# Autodesk Inventor assembly: Plataforma_robots
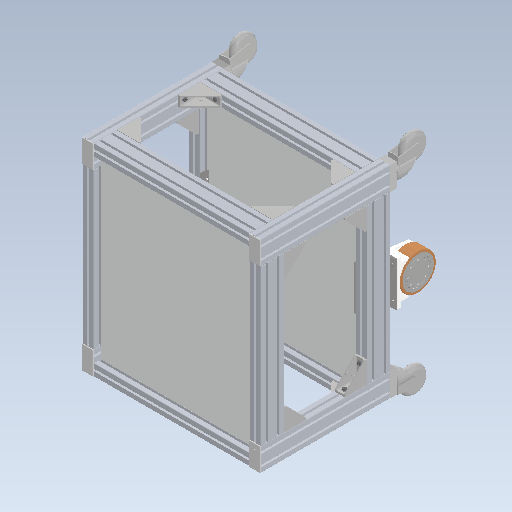
[picture p0: Inventor's stored thumbnail of the model, 512x512]
Saved by Autodesk Inventor 2021 (Build 250183000, 183)
## iProperties
Created: 2020-10-29
Part Number: Plataforma_robots
Document SubType Name: Assembly
Designer: German Di Fonzo
Author: German Di Fonzo
Title: Plataforma para Robots
## Documents named in this file (11)
- C:\Users\germi\OneDrive - Universidad Politécnica de Madrid\Escritorio\German Universidad\Master\Primer semestre\Diseño y Control de Robots\PECs\plataforma_robot\Plataforma_robots.iam
- C:\Users\germi\OneDrive - Universidad Politécnica de Madrid\Escritorio\German Universidad\Master\Primer semestre\Diseño y Control de Robots\PECs\plataforma_robot\Steps\perfil_45x90x600.ipt
- C:\Users\germi\OneDrive - Universidad Politécnica de Madrid\Escritorio\German Universidad\Master\Primer semestre\Diseño y Control de Robots\PECs\plataforma_robot\Steps\perfil_45x90x500.ipt
- C:\Users\germi\OneDrive - Universidad Politécnica de Madrid\Escritorio\German Universidad\Master\Primer semestre\Diseño y Control de Robots\PECs\plataforma_robot\piso1.ipt
- C:\Users\germi\OneDrive - Universidad Politécnica de Madrid\Escritorio\German Universidad\Master\Primer semestre\Diseño y Control de Robots\PECs\plataforma_robot\piso2.ipt
- C:\Users\germi\OneDrive - Universidad Politécnica de Madrid\Escritorio\German Universidad\Master\Primer semestre\Diseño y Control de Robots\PECs\plataforma_robot\Pletina (1).ipt
- C:\Users\germi\OneDrive - Universidad Politécnica de Madrid\Escritorio\German Universidad\Master\Primer semestre\Diseño y Control de Robots\PECs\plataforma_robot\Steps\tapa_superior.ipt
- C:\Users\germi\OneDrive - Universidad Politécnica de Madrid\Escritorio\German Universidad\Master\Primer semestre\Diseño y Control de Robots\PECs\plataforma_robot\Steps\L_45x90.ipt
- C:\Users\germi\OneDrive - Universidad Politécnica de Madrid\Escritorio\German Universidad\Master\Primer semestre\Diseño y Control de Robots\PECs\plataforma_robot\Steps\rueda_motriz.ipt
- C:\Users\germi\OneDrive - Universidad Politécnica de Madrid\Escritorio\German Universidad\Master\Primer semestre\Diseño y Control de Robots\PECs\plataforma_robot\Steps\castor.ipt
- C:\Users\germi\OneDrive - Universidad Politécnica de Madrid\Escritorio\German Universidad\Master\Primer semestre\Diseño y Control de Robots\PECs\plataforma_robot\sujecion_castor.ipt
## Components (46 placed, 10 different names)
1. perfil_45x90x600:1 — Coincidencia:1, Nivelación:1, Nivelación:2, Coincidencia:8, Nivelación:16, Nivelación:17, Coincidencia:19, Nivelación:38, Coincidencia:25, Nivelación:42, Coincidencia:45, Coincidencia:47
2. perfil_45x90x600:2 — Coincidencia:5, Nivelación:9, Nivelación:10, Coincidencia:7, Nivelación:14, Nivelación:15, Coincidencia:20, Nivelación:40, Coincidencia:22, Nivelación:41, Coincidencia:37, Coincidencia:49
3. perfil_45x90x600:3 — Coincidencia:9, Coincidencia:10, Nivelación:18, Nivelación:19, Nivelación:20, Nivelación:21, Nivelación:39, Coincidencia:41, Coincidencia:43
4. perfil_45x90x600:4 — Coincidencia:2, Nivelación:3, Nivelación:4, Nivelación:12, Coincidencia:6, Nivelación:13, Coincidencia:21, Coincidencia:39, Coincidencia:51
5. perfil_45x90x500:1 — Coincidencia:5, Nivelación:9, Nivelación:10, Coincidencia:9, Nivelación:18, Nivelación:21, Coincidencia:12, Nivelación:22, Nivelación:25, Coincidencia:17, Nivelación:34, Nivelación:36, Coincidencia:33, Nivelación:46, Nivelación:47, Coincidencia:40, Nivelación:54, Coincidencia:48, Nivelación:58, Coincidencia:55, Nivelación:61, Coincidencia:56, Nivelación:62, Coincidencia:74, Nivelación:78, Nivelación:79
6. perfil_45x90x500:2 — Coincidencia:8, Nivelación:16, Nivelación:17, Coincidencia:10, Nivelación:19, Nivelación:20, Coincidencia:14, Nivelación:26, Nivelación:29, Coincidencia:18, Nivelación:35, Nivelación:37, Coincidencia:34, Nivelación:48, Nivelación:49, Coincidencia:42, Nivelación:55, Coincidencia:46, Nivelación:57, Coincidencia:59, Nivelación:63, Coincidencia:63, Nivelación:65, Coincidencia:72, Nivelación:74, Nivelación:75
7. perfil_45x90x500:3 — Coincidencia:1, Nivelación:1, Nivelación:2, Coincidencia:2, Nivelación:3, Nivelación:4, Coincidencia:13, Nivelación:27, Nivelación:28, Coincidencia:16, Nivelación:30, Nivelación:33, Coincidencia:35, Nivelación:50, Nivelación:51, Coincidencia:44, Nivelación:56, Coincidencia:50, Nivelación:59, Coincidencia:60, Nivelación:64, Coincidencia:64, Nivelación:66, Coincidencia:70, Nivelación:72, Nivelación:73
8. perfil_45x90x500:4 — Nivelación:12, Coincidencia:6, Nivelación:13, Coincidencia:7, Nivelación:14, Nivelación:15, Coincidencia:11, Nivelación:23, Nivelación:24, Coincidencia:15, Nivelación:31, Nivelación:32, Coincidencia:32, Nivelación:44, Nivelación:45, Coincidencia:36, Nivelación:52, Coincidencia:38, Nivelación:53, Coincidencia:52, Coincidencia:66, Nivelación:67, Coincidencia:73, Nivelación:76, Nivelación:77
9. perfil_45x90x600:5 — Coincidencia:15, Coincidencia:16, Nivelación:30, Nivelación:31, Nivelación:32, Nivelación:33, Coincidencia:31, Coincidencia:65, Coincidencia:67
10. perfil_45x90x600:6 — Coincidencia:13, Coincidencia:14, Nivelación:26, Nivelación:27, Nivelación:28, Nivelación:29, Coincidencia:28, Coincidencia:61, Coincidencia:62
11. perfil_45x90x600:7 — Coincidencia:11, Coincidencia:12, Nivelación:22, Nivelación:23, Nivelación:24, Nivelación:25, Coincidencia:29, Nivelación:43, Coincidencia:53, Nivelación:60, Coincidencia:54
12. perfil_45x90x600:8 — Coincidencia:17, Coincidencia:18, Nivelación:34, Nivelación:35, Nivelación:36, Nivelación:37, Coincidencia:30, Coincidencia:57, Coincidencia:58
13. piso1:2 — Coincidencia:19, Coincidencia:20, Nivelación:38, Nivelación:39, Nivelación:40, Coincidencia:21, Coincidencia:23, Coincidencia:24, Coincidencia:26, Coincidencia:27
14. piso2:3 — Coincidencia:28, Coincidencia:29, Coincidencia:30, Coincidencia:31, Nivelación:43
15. Pletina (1):1 — Coincidencia:22, Coincidencia:23, Coincidencia:24, Nivelación:41, Coincidencia:69, Nivelación:70, Nivelación:71
16. Pletina (1):2 — Coincidencia:25, Coincidencia:26, Coincidencia:27, Nivelación:42, Coincidencia:68, Nivelación:68, Nivelación:69
17. tapa_superior:1 — Coincidencia:32, Nivelación:44, Nivelación:45
18. tapa_superior:2 — Coincidencia:33, Nivelación:46, Nivelación:47
19. tapa_superior:3 — Coincidencia:34, Nivelación:48, Nivelación:49
20. tapa_superior:4 — Coincidencia:35, Nivelación:50, Nivelación:51
21. L_45x90:1 — Coincidencia:46, Nivelación:57, Coincidencia:47
22. L_45x90:2 — Coincidencia:44, Coincidencia:45, Nivelación:56
23. L_45x90:3 — Coincidencia:50, Coincidencia:51, Nivelación:59
24. L_45x90:4 — Coincidencia:38, Coincidencia:39, Nivelación:53
25. L_45x90:5 — Coincidencia:36, Coincidencia:37, Nivelación:52
26. L_45x90:6 — Coincidencia:48, Coincidencia:49, Nivelación:58
27. L_45x90:7 — Coincidencia:40, Coincidencia:41, Nivelación:54
28. L_45x90:8 — Coincidencia:42, Coincidencia:43, Nivelación:55
29. L_45x90:9 — Coincidencia:62, Coincidencia:63, Nivelación:65
30. L_45x90:10 — Coincidencia:54, Coincidencia:55, Nivelación:61
31. L_45x90:11 — Coincidencia:60, Coincidencia:61, Nivelación:64
32. L_45x90:12 — Coincidencia:52, Coincidencia:53, Nivelación:60
33. L_45x90:13 — Coincidencia:56, Coincidencia:57, Nivelación:62
34. L_45x90:14 — Coincidencia:66, Coincidencia:67, Nivelación:67
35. L_45x90:15 — Coincidencia:58, Coincidencia:59, Nivelación:63
36. L_45x90:16 — Coincidencia:64, Coincidencia:65, Nivelación:66
37. rueda_motriz:1 — Coincidencia:69, Nivelación:70, Nivelación:71
38. rueda_motriz:2 — Coincidencia:68, Nivelación:68, Nivelación:69
39. sujecion_castor:1 — Coincidencia:70, Nivelación:72, Nivelación:73, De rotación:1
40. sujecion_castor:2 — Coincidencia:72, Nivelación:74, Nivelación:75, De rotación:2
41. sujecion_castor:3 — Coincidencia:74, Nivelación:78, Nivelación:79, De rotación:4
42. sujecion_castor:4 — Coincidencia:73, Nivelación:76, Nivelación:77, De rotación:3
43. castor:1 — De rotación:1
44. castor:2 — De rotación:3
45. castor:3 — De rotación:4
46. castor:4 — De rotación:2
## Relationships (149: Flush 74, Mate 71, RevoluteJoint 4)
- Coincidencia:1 [Mate]: perfil_45x90x600:1 ↔ perfil_45x90x500:3
- Nivelación:1 [Flush]: perfil_45x90x600:1 ↔ perfil_45x90x500:3
- Nivelación:2 [Flush]: perfil_45x90x600:1 ↔ perfil_45x90x500:3
- Coincidencia:2 [Mate]: perfil_45x90x600:4 ↔ perfil_45x90x500:3
- Nivelación:3 [Flush]: perfil_45x90x600:4 ↔ perfil_45x90x500:3
- Nivelación:4 [Flush]: perfil_45x90x600:4 ↔ perfil_45x90x500:3
- Coincidencia:5 [Mate]: perfil_45x90x600:2 ↔ perfil_45x90x500:1
- Nivelación:9 [Flush]: perfil_45x90x600:2 ↔ perfil_45x90x500:1
- Nivelación:10 [Flush]: perfil_45x90x600:2 ↔ perfil_45x90x500:1
- Nivelación:12 [Flush]: perfil_45x90x600:4 ↔ perfil_45x90x500:4
- Coincidencia:6 [Mate]: perfil_45x90x600:4 ↔ perfil_45x90x500:4
- Nivelación:13 [Flush]: perfil_45x90x600:4 ↔ perfil_45x90x500:4
- Coincidencia:7 [Mate]: perfil_45x90x600:2 ↔ perfil_45x90x500:4
- Nivelación:14 [Flush]: perfil_45x90x600:2 ↔ perfil_45x90x500:4
- Nivelación:15 [Flush]: perfil_45x90x600:2 ↔ perfil_45x90x500:4
- Coincidencia:8 [Mate]: perfil_45x90x600:1 ↔ perfil_45x90x500:2
- Nivelación:16 [Flush]: perfil_45x90x600:1 ↔ perfil_45x90x500:2
- Nivelación:17 [Flush]: perfil_45x90x600:1 ↔ perfil_45x90x500:2
- Coincidencia:9 [Mate]: perfil_45x90x600:3 ↔ perfil_45x90x500:1
- Coincidencia:10 [Mate]: perfil_45x90x600:3 ↔ perfil_45x90x500:2
- Nivelación:18 [Flush]: perfil_45x90x600:3 ↔ perfil_45x90x500:1
- Nivelación:19 [Flush]: perfil_45x90x600:3 ↔ perfil_45x90x500:2
- Nivelación:20 [Flush]: perfil_45x90x600:3 ↔ perfil_45x90x500:2
- Nivelación:21 [Flush]: perfil_45x90x600:3 ↔ perfil_45x90x500:1
- Coincidencia:11 [Mate]: perfil_45x90x500:4 ↔ perfil_45x90x600:7
- Coincidencia:12 [Mate]: perfil_45x90x500:1 ↔ perfil_45x90x600:7
- Nivelación:22 [Flush]: perfil_45x90x500:1 ↔ perfil_45x90x600:7
- Nivelación:23 [Flush]: perfil_45x90x500:4 ↔ perfil_45x90x600:7
- Nivelación:24 [Flush]: perfil_45x90x500:4 ↔ perfil_45x90x600:7
- Nivelación:25 [Flush]: perfil_45x90x500:1 ↔ perfil_45x90x600:7
- Coincidencia:13 [Mate]: perfil_45x90x500:3 ↔ perfil_45x90x600:6
- Coincidencia:14 [Mate]: perfil_45x90x500:2 ↔ perfil_45x90x600:6
- Nivelación:26 [Flush]: perfil_45x90x500:2 ↔ perfil_45x90x600:6
- Nivelación:27 [Flush]: perfil_45x90x500:3 ↔ perfil_45x90x600:6
- Nivelación:28 [Flush]: perfil_45x90x500:3 ↔ perfil_45x90x600:6
- Nivelación:29 [Flush]: perfil_45x90x500:2 ↔ perfil_45x90x600:6
- Coincidencia:15 [Mate]: perfil_45x90x500:4 ↔ perfil_45x90x600:5
- Coincidencia:16 [Mate]: perfil_45x90x500:3 ↔ perfil_45x90x600:5
- Nivelación:30 [Flush]: perfil_45x90x500:3 ↔ perfil_45x90x600:5
- Nivelación:31 [Flush]: perfil_45x90x500:4 ↔ perfil_45x90x600:5
- Nivelación:32 [Flush]: perfil_45x90x500:4 ↔ perfil_45x90x600:5
- Nivelación:33 [Flush]: perfil_45x90x500:3 ↔ perfil_45x90x600:5
- Coincidencia:17 [Mate]: perfil_45x90x500:1 ↔ perfil_45x90x600:8
- Coincidencia:18 [Mate]: perfil_45x90x500:2 ↔ perfil_45x90x600:8
- Nivelación:34 [Flush]: perfil_45x90x500:1 ↔ perfil_45x90x600:8
- Nivelación:35 [Flush]: perfil_45x90x500:2 ↔ perfil_45x90x600:8
- Nivelación:36 [Flush]: perfil_45x90x500:1 ↔ perfil_45x90x600:8
- Nivelación:37 [Flush]: perfil_45x90x500:2 ↔ perfil_45x90x600:8
- Coincidencia:19 [Mate]: perfil_45x90x600:1 ↔ piso1:2
- Coincidencia:20 [Mate]: perfil_45x90x600:2 ↔ piso1:2
- Nivelación:38 [Flush]: perfil_45x90x600:1 ↔ piso1:2
- Nivelación:39 [Flush]: perfil_45x90x600:3 ↔ piso1:2
- Nivelación:40 [Flush]: perfil_45x90x600:2 ↔ piso1:2
- Coincidencia:21 [Mate]: perfil_45x90x600:4 ↔ piso1:2
- Coincidencia:22 [Mate]: perfil_45x90x600:2 ↔ Pletina (1):1
- Coincidencia:23 [Mate]: piso1:2 ↔ Pletina (1):1
- Coincidencia:24 [Mate]: piso1:2 ↔ Pletina (1):1
- Nivelación:41 [Flush]: perfil_45x90x600:2 ↔ Pletina (1):1
- Coincidencia:25 [Mate]: perfil_45x90x600:1 ↔ Pletina (1):2
- Coincidencia:26 [Mate]: piso1:2 ↔ Pletina (1):2
- Coincidencia:27 [Mate]: piso1:2 ↔ Pletina (1):2
- Nivelación:42 [Flush]: perfil_45x90x600:1 ↔ Pletina (1):2
- Coincidencia:28 [Mate]: perfil_45x90x600:6 ↔ piso2:3
- Coincidencia:29 [Mate]: perfil_45x90x600:7 ↔ piso2:3
- Coincidencia:30 [Mate]: perfil_45x90x600:8 ↔ piso2:3
- Coincidencia:31 [Mate]: perfil_45x90x600:5 ↔ piso2:3
- Nivelación:43 [Flush]: perfil_45x90x600:7 ↔ piso2:3
- Coincidencia:32 [Mate]: perfil_45x90x500:4 ↔ tapa_superior:1
- Nivelación:44 [Flush]: perfil_45x90x500:4 ↔ tapa_superior:1
- Nivelación:45 [Flush]: perfil_45x90x500:4 ↔ tapa_superior:1
- Coincidencia:33 [Mate]: perfil_45x90x500:1 ↔ tapa_superior:2
- Nivelación:46 [Flush]: perfil_45x90x500:1 ↔ tapa_superior:2
- Nivelación:47 [Flush]: perfil_45x90x500:1 ↔ tapa_superior:2
- Coincidencia:34 [Mate]: perfil_45x90x500:2 ↔ tapa_superior:3
- Nivelación:48 [Flush]: perfil_45x90x500:2 ↔ tapa_superior:3
- Nivelación:49 [Flush]: perfil_45x90x500:2 ↔ tapa_superior:3
- Coincidencia:35 [Mate]: perfil_45x90x500:3 ↔ tapa_superior:4
- Nivelación:50 [Flush]: perfil_45x90x500:3 ↔ tapa_superior:4
- Nivelación:51 [Flush]: perfil_45x90x500:3 ↔ tapa_superior:4
- Coincidencia:36 [Mate]: perfil_45x90x500:4 ↔ L_45x90:5
- Coincidencia:37 [Mate]: perfil_45x90x600:2 ↔ L_45x90:5
- Nivelación:52 [Flush]: perfil_45x90x500:4 ↔ L_45x90:5
- Coincidencia:38 [Mate]: perfil_45x90x500:4 ↔ L_45x90:4
- Coincidencia:39 [Mate]: perfil_45x90x600:4 ↔ L_45x90:4
- Nivelación:53 [Flush]: perfil_45x90x500:4 ↔ L_45x90:4
- Coincidencia:40 [Mate]: perfil_45x90x500:1 ↔ L_45x90:7
- Coincidencia:41 [Mate]: perfil_45x90x600:3 ↔ L_45x90:7
- Nivelación:54 [Flush]: perfil_45x90x500:1 ↔ L_45x90:7
- Coincidencia:42 [Mate]: perfil_45x90x500:2 ↔ L_45x90:8
- Coincidencia:43 [Mate]: perfil_45x90x600:3 ↔ L_45x90:8
- Nivelación:55 [Flush]: perfil_45x90x500:2 ↔ L_45x90:8
- Coincidencia:44 [Mate]: perfil_45x90x500:3 ↔ L_45x90:2
- Coincidencia:45 [Mate]: perfil_45x90x600:1 ↔ L_45x90:2
- Nivelación:56 [Flush]: perfil_45x90x500:3 ↔ L_45x90:2
- Coincidencia:46 [Mate]: perfil_45x90x500:2 ↔ L_45x90:1
- Nivelación:57 [Flush]: perfil_45x90x500:2 ↔ L_45x90:1
- Coincidencia:47 [Mate]: perfil_45x90x600:1 ↔ L_45x90:1
- Coincidencia:48 [Mate]: perfil_45x90x500:1 ↔ L_45x90:6
- Coincidencia:49 [Mate]: perfil_45x90x600:2 ↔ L_45x90:6
- Nivelación:58 [Flush]: perfil_45x90x500:1 ↔ L_45x90:6
- Coincidencia:50 [Mate]: perfil_45x90x500:3 ↔ L_45x90:3
- Coincidencia:51 [Mate]: perfil_45x90x600:4 ↔ L_45x90:3
- Nivelación:59 [Flush]: perfil_45x90x500:3 ↔ L_45x90:3
- Coincidencia:52 [Mate]: perfil_45x90x500:4 ↔ L_45x90:12
- Coincidencia:53 [Mate]: perfil_45x90x600:7 ↔ L_45x90:12
- Nivelación:60 [Flush]: perfil_45x90x600:7 ↔ L_45x90:12
- Coincidencia:54 [Mate]: perfil_45x90x600:7 ↔ L_45x90:10
- Coincidencia:55 [Mate]: perfil_45x90x500:1 ↔ L_45x90:10
- Nivelación:61 [Flush]: perfil_45x90x500:1 ↔ L_45x90:10
- Coincidencia:56 [Mate]: perfil_45x90x500:1 ↔ L_45x90:13
- Coincidencia:57 [Mate]: perfil_45x90x600:8 ↔ L_45x90:13
- Nivelación:62 [Flush]: perfil_45x90x500:1 ↔ L_45x90:13
- Coincidencia:58 [Mate]: perfil_45x90x600:8 ↔ L_45x90:15
- Coincidencia:59 [Mate]: perfil_45x90x500:2 ↔ L_45x90:15
- Nivelación:63 [Flush]: perfil_45x90x500:2 ↔ L_45x90:15
- Coincidencia:60 [Mate]: perfil_45x90x500:3 ↔ L_45x90:11
- Coincidencia:61 [Mate]: perfil_45x90x600:6 ↔ L_45x90:11
- Nivelación:64 [Flush]: perfil_45x90x500:3 ↔ L_45x90:11
- Coincidencia:62 [Mate]: perfil_45x90x600:6 ↔ L_45x90:9
- Coincidencia:63 [Mate]: perfil_45x90x500:2 ↔ L_45x90:9
- Nivelación:65 [Flush]: perfil_45x90x500:2 ↔ L_45x90:9
- Coincidencia:64 [Mate]: perfil_45x90x500:3 ↔ L_45x90:16
- Coincidencia:65 [Mate]: perfil_45x90x600:5 ↔ L_45x90:16
- Nivelación:66 [Flush]: perfil_45x90x500:3 ↔ L_45x90:16
- Coincidencia:66 [Mate]: perfil_45x90x500:4 ↔ L_45x90:14
- Coincidencia:67 [Mate]: perfil_45x90x600:5 ↔ L_45x90:14
- Nivelación:67 [Flush]: perfil_45x90x500:4 ↔ L_45x90:14
- Coincidencia:68 [Mate]: Pletina (1):2 ↔ rueda_motriz:2
- Nivelación:68 [Flush]: Pletina (1):2 ↔ rueda_motriz:2
- Nivelación:69 [Flush]: Pletina (1):2 ↔ rueda_motriz:2
- Coincidencia:69 [Mate]: Pletina (1):1 ↔ rueda_motriz:1
- Nivelación:70 [Flush]: Pletina (1):1 ↔ rueda_motriz:1
- Nivelación:71 [Flush]: Pletina (1):1 ↔ rueda_motriz:1
- Coincidencia:70 [Mate]: perfil_45x90x500:3 ↔ sujecion_castor:1
- Nivelación:72 [Flush]: perfil_45x90x500:3 ↔ sujecion_castor:1
- Nivelación:73 [Flush]: perfil_45x90x500:3 ↔ sujecion_castor:1
- Coincidencia:72 [Mate]: perfil_45x90x500:2 ↔ sujecion_castor:2
- Nivelación:74 [Flush]: perfil_45x90x500:2 ↔ sujecion_castor:2
- Nivelación:75 [Flush]: perfil_45x90x500:2 ↔ sujecion_castor:2
- Coincidencia:73 [Mate]: perfil_45x90x500:4 ↔ sujecion_castor:4
- Nivelación:76 [Flush]: perfil_45x90x500:4 ↔ sujecion_castor:4
- Nivelación:77 [Flush]: perfil_45x90x500:4 ↔ sujecion_castor:4
- Coincidencia:74 [Mate]: perfil_45x90x500:1 ↔ sujecion_castor:3
- Nivelación:78 [Flush]: perfil_45x90x500:1 ↔ sujecion_castor:3
- Nivelación:79 [Flush]: perfil_45x90x500:1 ↔ sujecion_castor:3
- De rotación:1 [RevoluteJoint]: sujecion_castor:1 ↔ castor:1
- De rotación:2 [RevoluteJoint]: sujecion_castor:2 ↔ castor:4
- De rotación:3 [RevoluteJoint]: sujecion_castor:4 ↔ castor:2
- De rotación:4 [RevoluteJoint]: sujecion_castor:3 ↔ castor:3
